# Autodesk Inventor assembly: REV-41-1600
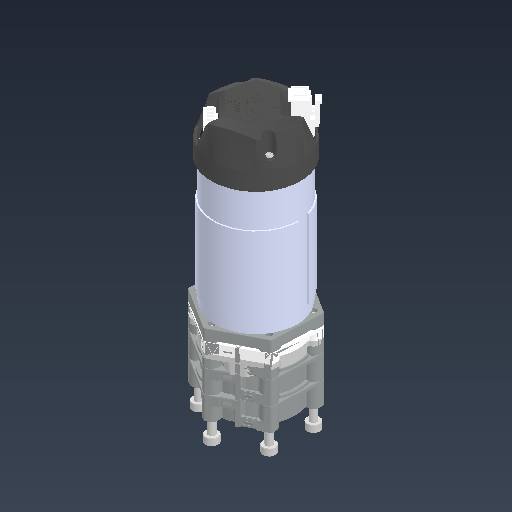
[picture p0: Inventor's stored thumbnail of the model, 512x512]
Saved by Autodesk Inventor 2026 (Build 300175000, 175)
## iProperties
Created: 2019-08-05
Part Number: REV-41-1600
Description: STEP AP214
Document SubType Name: Assembly
Designer: GameHD
Sending System: SolidWorks 2018
Preprocessor: SwSTEP 2.0
Title: REV-41-1600.STEP
Revision Number: ANY
## Documents named in this file (10)
- C:\Users\GameHD\Desktop\Phantom 16950\REV-41-1600\REV-41-1600.iam
- C:\Users\GameHD\Desktop\Phantom 16950\REV-41-1600\REV-41-1301 No Gearbox_Without Gearbox.iam
- C:\Users\GameHD\Desktop\Phantom 16950\REV-41-1600\REV-41-1607.ipt
- C:\Users\GameHD\Desktop\Phantom 16950\REV-41-1600\M3x8 Button Head_91239A113.ipt
- C:\Users\GameHD\Desktop\Phantom 16950\REV-41-1600\REV-41-1608.ipt
- C:\Users\GameHD\Desktop\Phantom 16950\REV-41-1600\REV-41-1603.iam
- C:\Users\GameHD\Desktop\Phantom 16950\REV-41-1600\REV-41-1602.iam
- C:\Users\GameHD\Desktop\Phantom 16950\REV-41-1600\REV-41-1601.iam
- C:\Users\GameHD\Desktop\Phantom 16950\REV-41-1600\REV-41-1604.iam
- C:\Users\GameHD\Desktop\Phantom 16950\REV-41-1600\M3X40_91290A136.ipt
## Components (15 placed, 15 different names)
1. REV-41-1301 No Gearbox_Without Gearbox_1 [sub-assembly]
2. REV-41-1607_2 — Совмещение:1, Совмещение:2, Совмещение:3
3. M3x8 Button Head_91239A113_3
4. REV-41-1608_4
5. REV-41-1603_5 [sub-assembly]
6. REV-41-1602_6 [sub-assembly]
7. REV-41-1601_7 [sub-assembly]
8. M3x8 Button Head_91239A113_8
9. REV-41-1604_9 [sub-assembly] — Совмещение:1, Совмещение:2, Совмещение:3
10. M3X40_91290A136_10
11. M3X40_91290A136_11
12. M3X40_91290A136_12
13. M3X40_91290A136_13
14. M3X40_91290A136_14
15. M3X40_91290A136_15
## Relationships (3: Mate 3)
- Совмещение:1 [Mate]: REV-41-1607_2 ↔ REV-41-1604_9
- Совмещение:2 [Mate]: REV-41-1607_2 ↔ REV-41-1604_9
- Совмещение:3 [Mate]: REV-41-1607_2 ↔ REV-41-1604_9
